# Autodesk Inventor assembly: FrontWheelForkAssembly
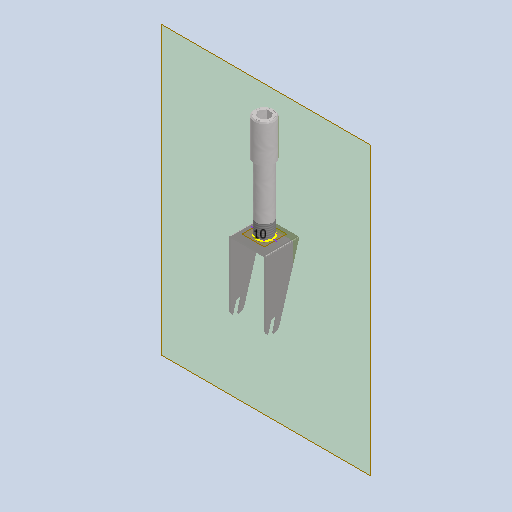
[picture p0: Inventor's stored thumbnail of the model, 512x512]
Saved by Autodesk Inventor 2022.2 (Build 262287010, 287A)
## iProperties
Created: 2022-04-13
Part Number: FrontWheelForkAssembly
Document SubType Name: Assembly
Designer: foriw
Mass: 127.99 g
Surface Area: 764.001 cm^2
Volume: 122.116 cm^3
Density: 1.0481 g/cm^3
Author: foriw
## Documents named in this file (6)
- C:\Users\Finn Oriwohl\Documents\htx\1g g\BeerCart-CAD-Inventor\Workspaces\Workspace\FrontWheelForkAssembly.iam
- C:\Users\Finn Oriwohl\Documents\htx\1g g\BeerCart-CAD-Inventor\Workspaces\Workspace\Solid2.ipt
- C:\Users\Finn Oriwohl\Documents\htx\1g g\BeerCart-CAD-Inventor\Workspaces\Workspace\Solid3.ipt
- C:\Users\Finn Oriwohl\Documents\htx\1g g\BeerCart-CAD-Inventor\Libraries\Content Center Files\en-US\ISO 4762(2)\ISO 4762 - M5 x 12ISO.ipt
- C:\Users\Finn Oriwohl\Documents\htx\1g g\BeerCart-CAD-Inventor\Libraries\Content Center Files\en-US\ISO 4762(2)\ISO 4762 - M5 x 8ISO.ipt
- C:\Users\Finn Oriwohl\Documents\htx\1g g\BeerCart-CAD-Inventor\Workspaces\Workspace\Fork lower hole plate.ipt
## Components (5 placed, 5 different names)
1. ForkUpperTube — Mate:1, Mate:3, Mate:5, Mate:6
2. ForkLowerTireMount — Mate:2, Mate:4, Mate:5, Mate:6
3. ISO 4762 M5 x 12:1 — Mate:1, Mate:2
4. ISO 4762 M5 x 8:1 — Mate:3, Mate:4
5. Fork lower hole plate:1
## Relationships (6: Mate 6)
- Mate:1: ForkUpperTube ↔ ISO 4762 M5 x 12:1
- Mate:2: ForkLowerTireMount ↔ ISO 4762 M5 x 12:1
- Mate:3: ForkUpperTube ↔ ISO 4762 M5 x 8:1
- Mate:4: ForkLowerTireMount ↔ ISO 4762 M5 x 8:1
- Mate:5: ForkUpperTube ↔ ForkLowerTireMount
- Mate:6: ForkUpperTube ↔ ForkLowerTireMount
